# Autodesk Inventor assembly: ddc final areoplane
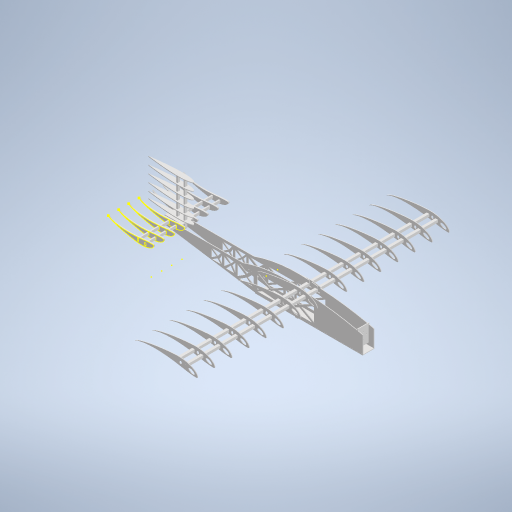
[picture p0: Inventor's stored thumbnail of the model, 512x512]
Saved by Autodesk Inventor 2024 (Build 280153000, 153)
## iProperties
Created: 2023-07-19
Part Number: ddc final areoplane
Document SubType Name: Assembly
Designer: USER
Author: USER
## Documents named in this file (13)
- C:\Users\USER\Desktop\ddc final areoplane.iam
- C:\Users\USER\Desktop\final side pannel.ipt
- C:\Users\USER\Desktop\New base.ipt
- C:\Users\USER\Desktop\wing rod.ipt
- C:\Users\USER\Desktop\new air foil.ipt
- C:\Users\USER\Desktop\new air foil_MIR.ipt
- C:\Users\USER\Desktop\motor mount.ipt
- C:\Users\USER\Desktop\tail horizontal rod.ipt
- C:\Users\USER\Desktop\horizontal air foil.ipt
- C:\Users\USER\Desktop\horizontal air foil_MIR.ipt
- C:\Users\USER\Desktop\tail plate.ipt
- C:\Users\USER\Desktop\tail vertical rod.ipt
- C:\Users\USER\Desktop\back side foil.ipt
## Components (41 placed, 12 different names)
1. final side pannel:1 — Mate:1, Mate:2, Mate:3, Mate:9, Symmetry:1, Mate:25, Mate:32, Mate:33
2. final side pannel:2 — Mate:4, Mate:5, Mate:6, Mate:7, Mate:8, Mate:10, Symmetry:1, Mate:18, Mate:19, Mate:20, Mate:21, Mate:22, Mate:23, Mate:24, Mate:31
3. New base:1 — Mate:1, Mate:2, Mate:3, Mate:4, Mate:5, Mate:6
4. wing rod:1 — Mate:7, Mate:8, Mate:12, Mate:13, Mate:14, Mate:15, Mate:17
5. wing rod:2 — Mate:9, Mate:10, Mate:11, Mate:16, Mate:49, Mate:50, Mate:51
6. new air foil:8 — Mate:16, Mate:17, Mate:18
7. motor mount:1 — Mate:19, Mate:20, Mate:21
8. tail horizontal rod:1 — Mate:22, Mate:23, Mate:26, Mate:28, Mate:29, Mate:30, Mate:52, Mate:53
9. tail horizontal rod:2 — Mate:24, Mate:25, Mate:27, Mate:54
10. tail plate:1 — Mate:31, Mate:32, Mate:33, Mate:37, Mate:38, Mate:39, Mate:40, Mate:41, Mate:42, Mate:48
11. tail vertical rod:1 — Mate:37, Mate:38, Mate:39, Mate:43, Mate:44, Mate:45, Mate:46, Mate:47
12. tail vertical rod:2 — Mate:40, Mate:41, Mate:42
13. back side foil:6 — Mate:46, Mate:47, Mate:48
14. new air foil:1 — Mate:13, Mate:14, Mate:15
15. new air foil:2
16. new air foil:3
17. new air foil:4
18. new air foil:5
19. new air foil:6
20. new air foil:7
21. horizontal air foil:1 — Mate:28, Mate:29, Mate:30
22. horizontal air foil:2
23. horizontal air foil:3
24. horizontal air foil:4
25. back side foil:1 — Mate:43, Mate:44, Mate:45
26. back side foil:2
27. back side foil:3
28. back side foil:4
29. back side foil:5
30. new air foil_MIR:8 — Mate:49, Mate:50, Mate:51
31. new air foil_MIR:9
32. new air foil_MIR:10
33. new air foil_MIR:11
34. new air foil_MIR:12
35. new air foil_MIR:13
36. new air foil_MIR:14
37. new air foil_MIR:15
38. horizontal air foil_MIR:4 — Mate:52, Mate:53, Mate:54
39. horizontal air foil_MIR:5
40. horizontal air foil_MIR:6
41. horizontal air foil_MIR:7
## Component patterns: (7 elements, first: new air foil:1), (4 elements, first: horizontal air foil:1), (5 elements, first: back side foil:1), (8 elements, first: new air foil_MIR:8), (4 elements, first: horizontal air foil_MIR:4)
## Relationships (52: Mate 51, Symmetry 1)
- Mate:1: final side pannel:1 ↔ New base:1
- Mate:2: final side pannel:1 ↔ New base:1
- Mate:3: final side pannel:1 ↔ New base:1
- Mate:4: final side pannel:2 ↔ New base:1
- Mate:5: final side pannel:2 ↔ New base:1
- Mate:6: final side pannel:2 ↔ New base:1
- Mate:7: final side pannel:2 ↔ wing rod:1
- Mate:8: final side pannel:2 ↔ wing rod:1
- Mate:9: final side pannel:1 ↔ wing rod:2
- Mate:10: final side pannel:2 ↔ wing rod:2
- Symmetry:1: final side pannel:1 ↔ final side pannel:2
- Mate:11 (-500 mm): wing rod:2
- Mate:12 (-500 mm): wing rod:1
- Mate:13: wing rod:1 ↔ new air foil:1
- Mate:14: wing rod:1 ↔ new air foil:1
- Mate:15: wing rod:1 ↔ new air foil:1
- Mate:16: wing rod:2 ↔ new air foil:8
- Mate:17: wing rod:1 ↔ new air foil:8
- Mate:18: final side pannel:2 ↔ new air foil:8
- Mate:19: final side pannel:2 ↔ motor mount:1
- Mate:20: final side pannel:2 ↔ motor mount:1
- Mate:21: final side pannel:2 ↔ motor mount:1
- Mate:22: final side pannel:2 ↔ tail horizontal rod:1
- Mate:23: final side pannel:2 ↔ tail horizontal rod:1
- Mate:24: final side pannel:2 ↔ tail horizontal rod:2
- Mate:25: final side pannel:1 ↔ tail horizontal rod:2
- Mate:26 (-150 mm): tail horizontal rod:1
- Mate:27 (-150 mm): tail horizontal rod:2
- Mate:28: tail horizontal rod:1 ↔ horizontal air foil:1
- Mate:29: tail horizontal rod:1 ↔ horizontal air foil:1
- Mate:30: tail horizontal rod:1 ↔ horizontal air foil:1
- Mate:31: final side pannel:2 ↔ tail plate:1
- Mate:32: final side pannel:1 ↔ tail plate:1
- Mate:33: final side pannel:1 ↔ tail plate:1
- Mate:37: tail plate:1 ↔ tail vertical rod:1
- Mate:38: tail plate:1 ↔ tail vertical rod:1
- Mate:39 (-150 mm): tail plate:1 ↔ tail vertical rod:1
- Mate:40: tail plate:1 ↔ tail vertical rod:2
- Mate:41: tail plate:1 ↔ tail vertical rod:2
- Mate:42 (-150 mm): tail plate:1 ↔ tail vertical rod:2
- Mate:43: tail vertical rod:1 ↔ back side foil:1
- Mate:44: tail vertical rod:1 ↔ back side foil:1
- Mate:45: tail vertical rod:1 ↔ back side foil:1
- Mate:46: tail vertical rod:1 ↔ back side foil:6
- Mate:47: tail vertical rod:1 ↔ back side foil:6
- Mate:48: tail plate:1 ↔ back side foil:6
- Mate:49: wing rod:2 ↔ new air foil_MIR:8
- Mate:50: wing rod:2 ↔ new air foil_MIR:8
- Mate:51: wing rod:2 ↔ new air foil_MIR:8
- Mate:52: tail horizontal rod:1 ↔ horizontal air foil_MIR:4
- Mate:53: tail horizontal rod:1 ↔ horizontal air foil_MIR:4
- Mate:54: tail horizontal rod:2 ↔ horizontal air foil_MIR:4
